# Autodesk Inventor assembly: 637112 servo block 25 spline
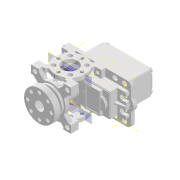
[picture p0: Inventor's stored thumbnail of the model, 180x180]
Saved by Autodesk Inventor 2020 (Build 240168000, 168)
## iProperties
Created: 2020-01-01
Part Number: 637112 servo block 25 spline
Document SubType Name: Assembly
Designer: ball
Author: ball
## Documents named in this file (6)
- C:\FTC\FTC8863CAD\Actobotics\637 parts\637112 servo block 25 spline.iam
- C:\FTC\FTC8863CAD\GoBilda\2000 Parts\2000-0025-0002.ipt
- C:\FTC\FTC8863CAD\Actobotics\575 parts\575112.ipt
- C:\FTC\FTC8863CAD\Actobotics\545 parts\545420.ipt
- C:\FTC\FTC8863CAD\Actobotics\535 parts\535118 assembly.ipt
- C:\FTC\FTC8863CAD\Actobotics\525 parts\525123.ipt
## Components (6 placed, 5 different names)
1. 2000-0025-0002:1 — Mate:1, Flush:1, Flush:2, Mate:13
2. 575112:1 — Mate:1, Flush:1, Flush:2, Mate:2, Mate:3, Mate:4, Mate:5, Mate:6, Mate:7
3. 545420:1 — Mate:2, Mate:3, Mate:4, Mate:8, Mate:10
4. 545420:2 — Mate:5, Mate:6, Mate:7, Mate:9, Mate:11
5. 535118 assembly:2 — Mate:8, Mate:9, Mate:10, Mate:11, Mate:12
6. 525123:1 — Mate:12, Mate:13
## Relationships (15: Mate 13, Flush 2)
- Mate:1: 2000-0025-0002:1 ↔ 575112:1
- Flush:1: 2000-0025-0002:1 ↔ 575112:1
- Flush:2: 2000-0025-0002:1 ↔ 575112:1
- Mate:2: 575112:1 ↔ 545420:1
- Mate:3: 575112:1 ↔ 545420:1
- Mate:4: 575112:1 ↔ 545420:1
- Mate:5: 575112:1 ↔ 545420:2
- Mate:6: 575112:1 ↔ 545420:2
- Mate:7: 575112:1 ↔ 545420:2
- Mate:8: 545420:1 ↔ 535118 assembly:2
- Mate:9: 545420:2 ↔ 535118 assembly:2
- Mate:10: 545420:1 ↔ 535118 assembly:2
- Mate:11: 545420:2 ↔ 535118 assembly:2
- Mate:12: 535118 assembly:2 ↔ 525123:1
- Mate:13: 2000-0025-0002:1 ↔ 525123:1
